# Autodesk Inventor assembly: ASY BSH tank frame
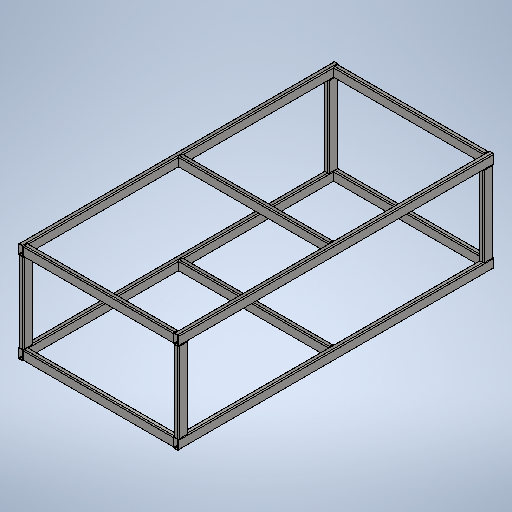
[picture p0: Inventor's stored thumbnail of the model, 512x512]
Saved by Autodesk Inventor 2025 (Build 290162010, 162A)
## iProperties
_SolveAssemblyDoc: Frame Generator Solve Assembly
_Version: 25.0.0
Created: 2024-09-22
Part Number: ASY BSH tank frame
Document SubType Name: Assembly
Designer: admin
Author: admin
## Documents named in this file (3)
- C:\Users\admin\YandexDisk-badmisterfox\домашниий пк\Inventor\BSH_Beshkino_bio_tank\ASY BSH tank frame.iam
- C:\Users\admin\YandexDisk-badmisterfox\домашниий пк\Inventor\BSH_Beshkino_bio_tank\BSH 601 Tank frame.ipt
- C:\Users\admin\YandexDisk-badmisterfox\домашниий пк\Inventor\BSH_Beshkino_bio_tank\ASY BSH tank frame\Frame\Frame 1727017497987.iam
## Components (2 placed, 2 different names)
1. BSH 601 Tank frame:1 — Flush:1, Flush:2, Mate:4
2. Frame 1727017497987:1 [sub-assembly]
## Relationships (3: Flush 2, Mate 1)
- Flush:1: BSH 601 Tank frame:1
- Flush:2: BSH 601 Tank frame:1
- Mate:4: BSH 601 Tank frame:1
